# Autodesk Inventor assembly: roller wheels
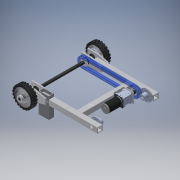
[picture p0: Inventor's stored thumbnail of the model, 180x180]
Saved by Autodesk Inventor 2016 (Build 200138000, 138)
## iProperties
Created: 2016-01-17
Part Number: roller wheels
Document SubType Name: Assembly
Designer: gus
Mass: 2632.89 g
Surface Area: 5756.22 cm^2
Volume: 1042.22 cm^3
Density: 2.52623 g/cm^3
Author: gus
## Documents named in this file (14)
- C:\Users\zachary\Downloads\robotfeb03\1510-stronghold-CAD-master\roller wheels\roller wheels.iam
- C:\Users\zachary\Downloads\robotfeb03\1510-stronghold-CAD-master\roller wheels\1x1x12.ipt
- C:\Users\zachary\Downloads\robotfeb03\1510-stronghold-CAD-master\roller wheels\am-0096a+500+Hex+Hub+r2.ipt
- C:\Users\zachary\Downloads\robotfeb03\1510-stronghold-CAD-master\roller wheels\1x1x10.ipt
- C:\Users\zachary\Downloads\robotfeb03\1510-stronghold-CAD-master\roller wheels\BAG motor\VersaPlanetary-1-Stage-with-BAG-Motor.iam
- C:\Users\zachary\Downloads\robotfeb03\1510-stronghold-CAD-master\roller wheels\217-2662-STEP-20140807.ipt
- C:\Users\zachary\Downloads\robotfeb03\1510-stronghold-CAD-master\roller wheels\BAG motor bracket.ipt
- C:\Users\zachary\Downloads\robotfeb03\1510-stronghold-CAD-master\roller wheels\Wheel Gusset.ipt
- C:\Users\zachary\Downloads\robotfeb03\1510-stronghold-CAD-master\roller wheels\hex bearing.ipt
- C:\Users\zachary\Downloads\robotfeb03\1510-stronghold-CAD-master\roller wheels\hex axle.ipt
- C:\Users\zachary\Downloads\robotfeb03\1510-stronghold-CAD-master\roller wheels\pnumatic wheel\PneumaticWheel_am-0970-2.iam
- C:\Users\zachary\Downloads\robotfeb03\1510-stronghold-CAD-master\roller wheels\roller wheels\Design Accelerator\Chain Drive1.iam
- C:\Users\zachary\Downloads\robotfeb03\1510-stronghold-CAD-master\roller wheels\shaft collar -hex.ipt
- C:\Users\zachary\Downloads\robotfeb03\1510-stronghold-CAD-master\roller cage\thumb block.ipt
## Components (25 placed, 13 different names)
1. 1x1x12:1 — Mate:5, Mate:6, Mate:7, Flush:1, Mate:8, Flush:2, Flush:4, Flush:7, Mate:13, Mate:14, Mate:18, Mate:19, Mate:20
2. 1x1x12:2 — Mate:1, Mate:3, Mate:4, Flush:1, Mate:8, Flush:2, Flush:3, Mate:15, Mate:16, Mate:17, Mate:21, Mate:22, Mate:23, Mate:34, Flush:11
3. am-0096a+500+Hex+Hub+r2:1 — Mate:1, Mate:3, Mate:4
4. am-0096a+500+Hex+Hub+r2:2 — Mate:5, Mate:6, Mate:7
5. 1x1x10:1 — Flush:3, Flush:4, Mate:9, Flush:5, Flush:11
6. VersaPlanetary-1-Stage-with-BAG-Motor:1 [sub-assembly] — Cylindrical:2, Mate:10, Mate:11, Mate:12, Flush:6
7. 217-2662-STEP-20140807:1 — Cylindrical:2, Flush:6, Mate:34
8. BAG motor bracket:1 — Mate:9, Flush:5, Mate:10, Mate:11, Mate:12
9. Wheel Gusset:1 — Flush:7, Mate:13, Mate:14, Rotational:4, Flush:13
10. Wheel Gusset:2 — Mate:18, Mate:19, Mate:20, Rotational:3, Flush:14, Flush:15
11. Wheel Gusset:3 — Mate:15, Mate:16, Mate:17, Rotational:2, Flush:16, Flush:17
12. Wheel Gusset:4 — Mate:21, Mate:22, Mate:23, Rotational:1, Mate:29, Mate:40
13. hex bearing:1 — Rotational:4, Flush:8, Flush:10, Slider:1, Mate:30
14. hex bearing:2 — Rotational:1, Flush:9
15. hex bearing:3 — Rotational:2, Flush:9, Flush:10, Mate:31
16. hex bearing:4 — Rotational:3, Flush:8
17. hex axle:1 — Slider:1, Mate:24, Mate:26, Mate:27, Mate:28, Mate:32, Mate:33, Mate:35, Mate:36, Mate:38, Mate:39, Flush:12
18. PneumaticWheel_am-0970-2:1 [sub-assembly] — Mate:26, Mate:27, Mate:29
19. PneumaticWheel_am-0970-2:2 [sub-assembly] — Mate:24, Mate:28, Mate:30, Mate:37
20. 217-2662-STEP-20140807:2 — Mate:31, Mate:32, Mate:33
21. Chain Drive:1 [sub-assembly]
22. shaft collar -hex:1 — Mate:35, Mate:36, Mate:37, Flush:12
23. shaft collar -hex:2 — Mate:38, Mate:39
24. thumb block:1 — Flush:13, Flush:14, Flush:15
25. thumb block:2 — Mate:40, Flush:16, Flush:17
## Relationships (61: Mate 38, Flush 17, RevoluteJoint 4, CylindricalJoint 1, TranslationJoint 1)
- Mate:1: 1x1x12:2 ↔ am-0096a+500+Hex+Hub+r2:1
- Mate:3: 1x1x12:2 ↔ am-0096a+500+Hex+Hub+r2:1
- Mate:4: 1x1x12:2 ↔ am-0096a+500+Hex+Hub+r2:1
- Mate:5: 1x1x12:1 ↔ am-0096a+500+Hex+Hub+r2:2
- Mate:6: 1x1x12:1 ↔ am-0096a+500+Hex+Hub+r2:2
- Mate:7: 1x1x12:1 ↔ am-0096a+500+Hex+Hub+r2:2
- Flush:1: 1x1x12:1 ↔ 1x1x12:2
- Mate:8 (254 mm): 1x1x12:1 ↔ 1x1x12:2
- Flush:2: 1x1x12:1 ↔ 1x1x12:2
- Flush:3: 1x1x12:2 ↔ 1x1x10:1
- Flush:4: 1x1x12:1 ↔ 1x1x10:1
- Cylindrical:2: VersaPlanetary-1-Stage-with-BAG-Motor:1 ↔ 217-2662-STEP-20140807:1
- Mate:9: 1x1x10:1 ↔ BAG motor bracket:1
- Flush:5 (-12.7 mm): 1x1x10:1 ↔ BAG motor bracket:1
- Mate:10: VersaPlanetary-1-Stage-with-BAG-Motor:1 ↔ BAG motor bracket:1
- Mate:11: VersaPlanetary-1-Stage-with-BAG-Motor:1 ↔ BAG motor bracket:1
- Mate:12: VersaPlanetary-1-Stage-with-BAG-Motor:1 ↔ BAG motor bracket:1
- Flush:6: VersaPlanetary-1-Stage-with-BAG-Motor:1 ↔ 217-2662-STEP-20140807:1
- Flush:7: 1x1x12:1 ↔ Wheel Gusset:1
- Mate:13: 1x1x12:1 ↔ Wheel Gusset:1
- Mate:14: 1x1x12:1 ↔ Wheel Gusset:1
- Mate:15: 1x1x12:2 ↔ Wheel Gusset:3
- Mate:16: 1x1x12:2 ↔ Wheel Gusset:3
- Mate:17: 1x1x12:2 ↔ Wheel Gusset:3
- Mate:18: 1x1x12:1 ↔ Wheel Gusset:2
- Mate:19: 1x1x12:1 ↔ Wheel Gusset:2
- Mate:20: 1x1x12:1 ↔ Wheel Gusset:2
- Mate:21: 1x1x12:2 ↔ Wheel Gusset:4
- Mate:22: 1x1x12:2 ↔ Wheel Gusset:4
- Mate:23: 1x1x12:2 ↔ Wheel Gusset:4
- Rotational:1 [RevoluteJoint]: Wheel Gusset:4 ↔ hex bearing:2
- Rotational:2 [RevoluteJoint]: Wheel Gusset:3 ↔ hex bearing:3
- Rotational:3 [RevoluteJoint]: Wheel Gusset:2 ↔ hex bearing:4
- Rotational:4 [RevoluteJoint]: Wheel Gusset:1 ↔ hex bearing:1
- Flush:8: hex bearing:1 ↔ hex bearing:4
- Flush:9: hex bearing:2 ↔ hex bearing:3
- Flush:10: hex bearing:1 ↔ hex bearing:3
- Slider:1 [TranslationJoint]: hex bearing:1 ↔ hex axle:1
- Mate:24: hex axle:1 ↔ PneumaticWheel_am-0970-2:2
- Mate:26: hex axle:1 ↔ PneumaticWheel_am-0970-2:1
- Mate:27: hex axle:1 ↔ PneumaticWheel_am-0970-2:1
- Mate:28: hex axle:1 ↔ PneumaticWheel_am-0970-2:2
- Mate:29: Wheel Gusset:4 ↔ PneumaticWheel_am-0970-2:1
- Mate:30: hex bearing:1 ↔ PneumaticWheel_am-0970-2:2
- Mate:31: hex bearing:3 ↔ 217-2662-STEP-20140807:2
- Mate:32: hex axle:1 ↔ 217-2662-STEP-20140807:2
- Mate:33: hex axle:1 ↔ 217-2662-STEP-20140807:2
- Mate:34 (7.874 mm): 1x1x12:2 ↔ 217-2662-STEP-20140807:1
- Flush:11 (101.6 mm): 1x1x12:2 ↔ 1x1x10:1
- Mate:35: hex axle:1 ↔ shaft collar -hex:1
- Mate:36: hex axle:1 ↔ shaft collar -hex:1
- Mate:37: PneumaticWheel_am-0970-2:2 ↔ shaft collar -hex:1
- Mate:38: hex axle:1 ↔ shaft collar -hex:2
- Mate:39: hex axle:1 ↔ shaft collar -hex:2
- Flush:12: hex axle:1 ↔ shaft collar -hex:1
- Flush:13: Wheel Gusset:1 ↔ thumb block:1
- Flush:14: Wheel Gusset:2 ↔ thumb block:1
- Flush:15: Wheel Gusset:2 ↔ thumb block:1
- Mate:40: Wheel Gusset:4 ↔ thumb block:2
- Flush:16: Wheel Gusset:3 ↔ thumb block:2
- Flush:17: Wheel Gusset:3 ↔ thumb block:2
